# Autodesk Inventor assembly: ASY ДМФ 0100 Барабан v2.1
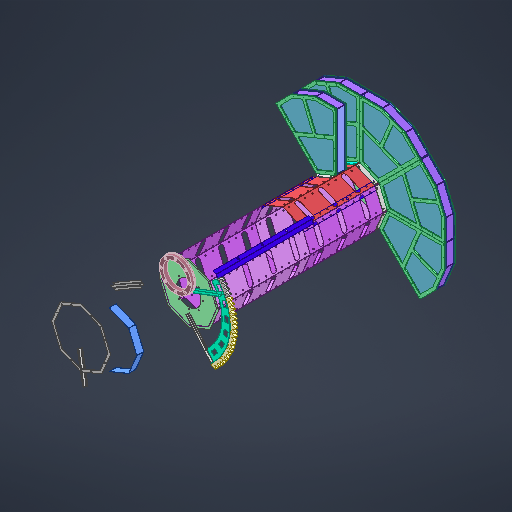
[picture p0: Inventor's stored thumbnail of the model, 512x512]
Saved by Autodesk Inventor 2026.2 (Build 302298000, 298)
## iProperties
Created: 2024-04-28
Part Number: ASY ДМФ 0100 Барабан v2.1
Document SubType Name: Assembly
Designer: pokla
Author: pokla
## Documents named in this file (26)
- C:\Users\admin\Documents\Inventor\DMF-Disk-Micro-Filter\Барабан v2.1\ASY ДМФ 0100 Барабан v2.1.iam
- C:\Users\admin\Documents\Inventor\DMF-Disk-Micro-Filter\Барабан v2.1\DMF 01 21 Барабан торец НОС v2.1.ipt
- C:\Users\admin\Documents\Inventor\DMF-Disk-Micro-Filter\Барабан v2.1\DMF 01 13 Барабан Лист лев брт v2.1.ipt
- C:\Users\admin\Documents\Inventor\DMF-Disk-Micro-Filter\Барабан v2.1\DMF 01 14 Барабан Лист прав брт v2.1.ipt
- C:\Users\admin\Documents\Inventor\DMF-Disk-Micro-Filter\Барабан v2.1\DMF 01 31 Барабан Опорное кольцо НОС v2.1.ipt
- C:\Users\admin\Documents\Inventor\DMF-Disk-Micro-Filter\Барабан v2.1\DMF 01 17 опора крышки v2.1.ipt
- C:\Users\admin\Documents\Inventor\DMF-Disk-Micro-Filter\Барабан v2.1\DMF 000 размеры v2.1.ipt
- C:\Users\admin\Documents\Inventor\DMF-Disk-Micro-Filter\Барабан v2.1\DMF 01 12 Барабан усилитель v2.1.ipt
- C:\Users\admin\Documents\Inventor\DMF-Disk-Micro-Filter\Барабан v2.1\ASY DMF 010 cap v2.1.iam
- C:\Users\admin\Documents\Inventor\DMF-Disk-Micro-Filter\Барабан v2.1\DMF 01 32 Барабан Опорное кольцо КОРМА v2.1.ipt
- C:\Users\admin\Documents\Inventor\DMF-Disk-Micro-Filter\Барабан v2.1\DMF 01 22 Барабан торец КОРМА v2.1.ipt
- C:\Users\admin\Documents\Inventor\DMF-Disk-Micro-Filter\Барабан v2.1\ASY DMF filter package v2.1.iam
- C:\Users\admin\Documents\Inventor\DMF-Disk-Micro-Filter\Барабан v2.1\DMF 01 21 cylinder butt end nose.ipt
- C:\Users\admin\Documents\Inventor\DMF-Disk-Micro-Filter\Барабан v2.1\DMF 2.1 01 43 Gear rim 3.ipt
- C:\Users\admin\Documents\Inventor\DMF-Disk-Micro-Filter\Барабан v2.1\DMF 2.1 01 44 Gear rim 4.ipt
- C:\Users\admin\Documents\Inventor\DMF-Disk-Micro-Filter\Барабан v2.1\DMF 2.1 01 45 Gear ring 5.ipt
- C:\Users\admin\Documents\Inventor\DMF-Disk-Micro-Filter\Барабан v2.1\DMF 2.1 01 46 Gear axis wheel 6.ipt
- C:\Users\admin\Documents\Inventor\DMF-Disk-Micro-Filter\Барабан v2.1\DMF 01 13 Барабан усилитель v2.1.ipt
- C:\Users\admin\Documents\Inventor\DMF-Disk-Micro-Filter\шестерни 06.09.2025\DMF sector big gear 2.1.ipt
- C:\Users\admin\Documents\Inventor\DMF-Disk-Micro-Filter\Барабан v2.1\DMF 01 15 drum sheet 1.ipt
- C:\Users\admin\Documents\Inventor\DMF-Disk-Micro-Filter\ДМФ 01 12 Барабан усилитель.ipt
- C:\Users\admin\Documents\Inventor\DMF-Disk-Micro-Filter\ДМФ 01 15 Барабан усилитель борта.ipt
- C:\Users\admin\Documents\Inventor\DMF-Disk-Micro-Filter\Барабан v2.1\DMF 2.1 Пластина паза маленькая.ipt
- C:\Users\admin\Documents\Inventor\DMF-Disk-Micro-Filter\Барабан v2.1\DMF 2.1 Пластина паза большая.ipt
- C:\Users\admin\Documents\Inventor\DMF-Disk-Micro-Filter\Барабан v2.1\DMF 01 17 опора крышки v2.1_CPY.ipt
- C:\Users\admin\Documents\Inventor\DMF-Disk-Micro-Filter\Барабан v2.1\DMF 01 11 cylinder sheet cap v2.1.ipt
## Components (44 placed, 30 different names)
1. DMF 000 размеры v2.1.ipt:1
2. DMF 01 21 Барабан торец НОС v2.1.ipt:1 — Rigid:101, Mate:49
3. DMF 01 31 Барабан Опорное кольцо НОС v2.1.ipt:1
4. DMF 01 32 Барабан Опорное кольцо КОРМА v2.1.ipt:1 — Rigid:20
5. DMF 01 22 Барабан торец КОРМА v2.1.ipt:1 — Rigid:20, Rigid:51, Rigid:53, Mate:36, Flush:22, Flush:23, Mate:37, Rigid:97, Mate:46
6. DMF 01 13 Барабан Лист лев брт v2.1.ipt:1 — Rigid:51, Rigid:98
7. DMF 01 14 Барабан Лист прав брт v2.1.ipt:1 — Rigid:53
8. DMF 01 17 опора крышки v2.1.ipt:1 — Mate:37, Mate:46, Mate:47, Mate:48
9. DMF 01 17 опора крышки v2.1.ipt:2 — Mate:36, Flush:22, Flush:23
10. DMF 01 11 cylinder sheet cap v2.1.ipt:1 — Mate:47, Rigid:100
11. ASY DMF 010 cap v2.1.iam:1 [sub-assembly]
12. DMF 01 21 cylinder butt end nose.ipt:1
13. DMF 2.1 01 45 Gear ring 5.ipt:1
14. DMF 2.1 01 46 Gear axis wheel 6.ipt:1
15. DMF 2.1 01 44 Gear rim 4.ipt:1 — Rigid:102, Rigid:110
16. DMF 2.1 01 43 Gear rim 3.ipt:2 — Rigid:102, Rigid:103, Rigid:109
17. DMF 01 15 drum sheet 1.ipt:1
18. ДМФ 01 12 Барабан усилитель.ipt:2 — Rigid:56, Rigid:57, Rigid:89
19. ДМФ 01 15 Барабан усилитель борта.ipt:3 — Rigid:56
20. ДМФ 01 15 Барабан усилитель борта.ipt:4 — Rigid:57
21. ДМФ 01 12 Барабан усилитель:3 — Rigid:89
22. ДМФ 01 15 Барабан усилитель борта:5
23. ДМФ 01 15 Барабан усилитель борта:6
24. DMF 01 17 опора крышки №2 v2.1:1
25. DMF 01 12 Барабан усилитель v2.1.ipt:1 — Rigid:82
26. DMF 01 13 Барабан усилитель v2.1.ipt:1 — Rigid:82
27. DMF 01 12 Барабан усилитель v2.1.ipt:2
28. DMF 01 13 Барабан усилитель v2.1.ipt:2 — Rigid:103
29. DMF 2.1 Пластина паза маленькая.ipt:1
30. DMF 2.1 Пластина паза большая:1 — Rigid:110, Mate:49
31. ASY DMF filter package v2.1.iam:1 [sub-assembly]
32. DMF sector big gear 2.1.ipt:1 — Rigid:104, Rigid:109
33. ASY DMF filter package v2.1:2 [sub-assembly]
34. ASY DMF filter package v2.1:3 [sub-assembly]
35. ASY DMF filter package v2.1:4 [sub-assembly]
36. DMF 01 13 Барабан Лист лев брт v2.1:2 — Rigid:97, Rigid:99, Mate:48
37. DMF 01 13 Барабан Лист лев брт v2.1:3 — Rigid:98
38. DMF 01 13 Барабан Лист лев брт v2.1:4 — Rigid:99, Rigid:101
39. DMF sector big gear 2.1:2 — Rigid:104, Rigid:105
40. DMF sector big gear 2.1:3 — Rigid:105, Rigid:106
41. DMF sector big gear 2.1:4 — Rigid:106, Rigid:107
42. DMF sector big gear 2.1:5 — Rigid:107, Rigid:108
43. DMF sector big gear 2.1:6 — Rigid:108
44. ASY DMF filter package v2.1:5 [sub-assembly] — Rigid:100
## Relationships (36: WeldJoint 25, Mate 7, Flush 4)
- Rigid:20 [WeldJoint]: DMF 01 32 Барабан Опорное кольцо КОРМА v2.1.ipt:1 ↔ DMF 01 22 Барабан торец КОРМА v2.1.ipt:1
- Rigid:51 [WeldJoint]: DMF 01 22 Барабан торец КОРМА v2.1.ipt:1 ↔ DMF 01 13 Барабан Лист лев брт v2.1.ipt:1
- Rigid:53 [WeldJoint]: DMF 01 22 Барабан торец КОРМА v2.1.ipt:1 ↔ DMF 01 14 Барабан Лист прав брт v2.1.ipt:1
- Mate:36: DMF 01 22 Барабан торец КОРМА v2.1.ipt:1 ↔ DMF 01 17 опора крышки v2.1.ipt:2
- Flush:22 (2 mm): DMF 01 22 Барабан торец КОРМА v2.1.ipt:1 ↔ DMF 01 17 опора крышки v2.1.ipt:2
- Flush:23 (2 mm): DMF 01 22 Барабан торец КОРМА v2.1.ipt:1 ↔ DMF 01 17 опора крышки v2.1.ipt:2
- Mate:37: DMF 01 22 Барабан торец КОРМА v2.1.ipt:1 ↔ DMF 01 17 опора крышки v2.1.ipt:1
- Rigid:56 [WeldJoint]: ДМФ 01 12 Барабан усилитель.ipt:2 ↔ ДМФ 01 15 Барабан усилитель борта.ipt:3
- Rigid:57 [WeldJoint]: ДМФ 01 12 Барабан усилитель.ipt:2 ↔ ДМФ 01 15 Барабан усилитель борта.ipt:4
- [Mate]: DMF 01 22 Барабан торец КОРМА v2.1.ipt:1 ↔ DMF 01 11 cylinder sheet cap v2.1.ipt:1
- [Flush]: DMF 01 22 Барабан торец КОРМА v2.1.ipt:1 ↔ DMF 01 11 cylinder sheet cap v2.1.ipt:1
- [Flush]: DMF 01 22 Барабан торец КОРМА v2.1.ipt:1 ↔ DMF 01 11 cylinder sheet cap v2.1.ipt:1
- Rigid:82 [WeldJoint]: DMF 01 12 Барабан усилитель v2.1.ipt:1 ↔ DMF 01 13 Барабан усилитель v2.1.ipt:1
- [WeldJoint]: ДМФ 01 12 Барабан усилитель:3 ↔ ДМФ 01 15 Барабан усилитель борта:5
- [WeldJoint]: ДМФ 01 12 Барабан усилитель:3 ↔ ДМФ 01 15 Барабан усилитель борта:6
- Rigid:89 [WeldJoint]: ДМФ 01 12 Барабан усилитель.ipt:2 ↔ ДМФ 01 12 Барабан усилитель:3
- [WeldJoint]: DMF 01 11 cylinder sheet cap v2.1.ipt:1 ↔ ASY DMF filter package v2.1.iam:1
- [WeldJoint]: DMF 01 11 cylinder sheet cap v2.1.ipt:1 ↔ ASY DMF filter package v2.1:2
- Rigid:97 [WeldJoint]: DMF 01 22 Барабан торец КОРМА v2.1.ipt:1 ↔ DMF 01 13 Барабан Лист лев брт v2.1:2
- Rigid:98 [WeldJoint]: DMF 01 13 Барабан Лист лев брт v2.1.ipt:1 ↔ DMF 01 13 Барабан Лист лев брт v2.1:3
- Rigid:99 [WeldJoint]: DMF 01 13 Барабан Лист лев брт v2.1:2 ↔ DMF 01 13 Барабан Лист лев брт v2.1:4
- Mate:46: DMF 01 22 Барабан торец КОРМА v2.1.ipt:1 ↔ DMF 01 17 опора крышки v2.1.ipt:1
- Mate:47: DMF 01 17 опора крышки v2.1.ipt:1 ↔ DMF 01 11 cylinder sheet cap v2.1.ipt:1
- Mate:48: DMF 01 17 опора крышки v2.1.ipt:1 ↔ DMF 01 13 Барабан Лист лев брт v2.1:2
- Rigid:100 [WeldJoint]: DMF 01 11 cylinder sheet cap v2.1.ipt:1 ↔ ASY DMF filter package v2.1:5
- Rigid:101 [WeldJoint]: DMF 01 21 Барабан торец НОС v2.1.ipt:1 ↔ DMF 01 13 Барабан Лист лев брт v2.1:4
- Rigid:102 [WeldJoint]: DMF 2.1 01 44 Gear rim 4.ipt:1 ↔ DMF 2.1 01 43 Gear rim 3.ipt:2
- Rigid:103 [WeldJoint]: DMF 2.1 01 43 Gear rim 3.ipt:2 ↔ DMF 01 13 Барабан усилитель v2.1.ipt:2
- Rigid:104 [WeldJoint]: DMF sector big gear 2.1.ipt:1 ↔ DMF sector big gear 2.1:2
- Rigid:105 [WeldJoint]: DMF sector big gear 2.1:2 ↔ DMF sector big gear 2.1:3
- Rigid:106 [WeldJoint]: DMF sector big gear 2.1:3 ↔ DMF sector big gear 2.1:4
- Rigid:107 [WeldJoint]: DMF sector big gear 2.1:4 ↔ DMF sector big gear 2.1:5
- Rigid:108 [WeldJoint]: DMF sector big gear 2.1:5 ↔ DMF sector big gear 2.1:6
- Rigid:109 [WeldJoint]: DMF 2.1 01 43 Gear rim 3.ipt:2 ↔ DMF sector big gear 2.1.ipt:1
- Rigid:110 [WeldJoint]: DMF 2.1 01 44 Gear rim 4.ipt:1 ↔ DMF 2.1 Пластина паза большая:1
- Mate:49 (120 mm): DMF 01 21 Барабан торец НОС v2.1.ipt:1 ↔ DMF 2.1 Пластина паза большая:1
## Named parameters: d460_d378 = 0 mm, d461_d379 = 0 mm
